# Autodesk Inventor assembly: Assembly_HoLiSheet_TwoHalf_v1
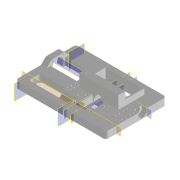
[picture p0: Inventor's stored thumbnail of the model, 180x180]
Saved by Autodesk Inventor 2022 (Build 260153000, 153)
## iProperties
Created: 2022-09-27
Part Number: Assembly_HoLiSheet_TwoHalf_v1
Document SubType Name: Assembly
Designer: UC2
Author: UC2
## Documents named in this file (3)
- C:\Users\diederichbenedict\Dropbox\Dokumente\Promotion\PROJECTS\HoLiSheet\INVENTOR\Assembly_HoLiSheet_TwoHalf_v1.iam
- C:\Users\diederichbenedict\Dropbox\Dokumente\Promotion\PROJECTS\HoLiSheet\INVENTOR\10_Wellplate_base_p2_v1.ipt
- C:\Users\diederichbenedict\Dropbox\Dokumente\Promotion\PROJECTS\HoLiSheet\INVENTOR\10_Wellplate_base_p1_v1.ipt
## Components (2 placed, 2 different names)
1. 10_Wellplate_base_p2_v1:1 — Passend:2, Fluchtend:1, Fluchtend:3
2. 10_Wellplate_base_p1_v1:1 — Passend:1, Passend:3, Fluchtend:2
## Relationships (6: Mate 3, Flush 3)
- Passend:1 [Mate]: 10_Wellplate_base_p1_v1:1
- Passend:2 [Mate]: 10_Wellplate_base_p2_v1:1
- Fluchtend:1 [Flush]: 10_Wellplate_base_p2_v1:1
- Passend:3 [Mate]: 10_Wellplate_base_p1_v1:1
- Fluchtend:2 [Flush]: 10_Wellplate_base_p1_v1:1
- Fluchtend:3 [Flush]: 10_Wellplate_base_p2_v1:1
